# Autodesk Inventor assembly: GPS-Compass_assembly
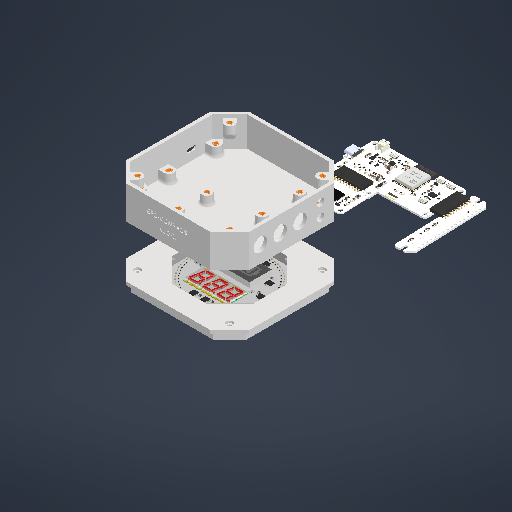
[picture p0: Inventor's stored thumbnail of the model, 512x512]
Saved by Autodesk Inventor 2026.1 (Build 301233020, 233B)
## iProperties
Created: 2025-11-19
Part Number: GPS-Compass_assembly
Document SubType Name: Assembly
Designer: MenMe
Author: MenMe
## Documents named in this file (10)
- C:\Users\MenMe\Documents\GitHub\GPS-Compass\Mechanical\GPS-Compass_assembly\GPS-Compass_assembly.iam
- C:\Users\MenMe\Documents\GitHub\GPS-Compass\Mechanical\GPS-Compass_assembly\GPS-Compass_box.ipt
- C:\Users\MenMe\Documents\GitHub\GPS-Compass\Mechanical\GPS-Compass_assembly\GPS-Compass_top.ipt
- C:\Users\MenMe\Documents\GitHub\GPS-Compass\Mechanical\PCB_3D_models\GPS-Compass_Arrow\GPS-Compass_Arrow\GPS-Compass_Arrow.iam
- C:\Users\MenMe\Documents\GitHub\GPS-Compass\Mechanical\GPS-Compass_assembly\GPS-Compass_plexi.ipt
- C:\Users\MenMe\Documents\GitHub\GPS-Compass\Mechanical\GPS-Compass_assembly\DODGE INSERT M3X4(D5-Dill4.8)\DODGE INSERT M3X4(D5-Dill4.8)\DODGE INSERT M3X4(D5-Dill4.8).ipt
- C:\Users\MenMe\Documents\Inventor\Content Center Files\R2026\en-US\ISO 4762(2)\ISO 4762 - M3 x 16ISO.ipt
- C:\Users\MenMe\Documents\GitHub\GPS-Compass\Mechanical\PCB_3D_models\GPS-Compass\GPS-Compass\GPS-Compass.ipt
- C:\Users\MenMe\Documents\GitHub\GPS-Compass\Mechanical\PCB_3D_models\GPS-Compass_UI\GPS-Compass_UI\GPS-Compass_UI.ipt
- C:\Users\MenMe\Documents\GitHub\GPS-Compass\Mechanical\GPS-Compass_GNSS\GPS-Compass_GNSS\GPS-Compass_GNSS.iam
## Components (24 placed, 9 different names)
1. GPS-Compass_box:1 — Mate:2, Mate:3, Mate:4, Insert:1, Insert:6, Insert:7, Insert:8, Insert:9, Mate:11, Insert:10, Insert:11, Insert:12, Insert:13, Insert:14, Insert:15, Insert:16
2. GPS-Compass_top:1 — Mate:2, Mate:3, Mate:4, Mate:5, Mate:6, Mate:7, Mate:8, Mate:9, Mate:10, Insert:2, Insert:3, Insert:4, Insert:5
3. GPS-Compass_Arrow:1 [sub-assembly] — Mate:5, Mate:6, Mate:7
4. GPS-Compass_plexi:1 — Mate:8, Mate:9, Mate:10
5. DODGE INSERT M3X4(D5-Dill4.8):1 — Insert:1
6. DODGE INSERT M3X4(D5-Dill4.8):2 — Insert:6
7. ISO 4762 M3 x 16:1 — Insert:2
8. ISO 4762 M3 x 16:2 — Insert:3
9. ISO 4762 M3 x 16:3 — Insert:4
10. ISO 4762 M3 x 16:4 — Insert:5
11. DODGE INSERT M3X4(D5-Dill4.8):3 — Insert:7
12. DODGE INSERT M3X4(D5-Dill4.8):4 — Insert:8
13. DODGE INSERT M3X4(D5-Dill4.8):5 — Insert:9
14. DODGE INSERT M3X4(D5-Dill4.8):6 — Mate:11
15. DODGE INSERT M3X4(D5-Dill4.8):7 — Insert:10
16. DODGE INSERT M3X4(D5-Dill4.8):8 — Insert:11
17. DODGE INSERT M3X4(D5-Dill4.8):9 — Insert:12
18. DODGE INSERT M3X4(D5-Dill4.8):10 — Insert:13
19. DODGE INSERT M3X4(D5-Dill4.8):11 — Insert:14
20. DODGE INSERT M3X4(D5-Dill4.8):12 — Insert:15
21. GPS-Compass:1 — Mate:13, Flush:3, Flush:4, Flush:5, Mate:14, Flush:6
22. DODGE INSERT M3X4(D5-Dill4.8):13 — Insert:16
23. GPS-Compass_UI:1 — Mate:13, Flush:3, Flush:6
24. GPS-Compass_GNSS:1 [sub-assembly] — Flush:4, Flush:5, Mate:14
## Relationships (32: Insert 16, Mate 12, Flush 4)
- Mate:2 (-80 mm): GPS-Compass_box:1 ↔ GPS-Compass_top:1
- Mate:3: GPS-Compass_box:1 ↔ GPS-Compass_top:1
- Mate:4: GPS-Compass_box:1 ↔ GPS-Compass_top:1
- Mate:5: GPS-Compass_top:1 ↔ GPS-Compass_Arrow:1
- Mate:6: GPS-Compass_top:1 ↔ GPS-Compass_Arrow:1
- Mate:7: GPS-Compass_top:1 ↔ GPS-Compass_Arrow:1
- Mate:8: GPS-Compass_top:1 ↔ GPS-Compass_plexi:1
- Mate:9: GPS-Compass_top:1 ↔ GPS-Compass_plexi:1
- Mate:10: GPS-Compass_top:1 ↔ GPS-Compass_plexi:1
- Insert:1: GPS-Compass_box:1 ↔ DODGE INSERT M3X4(D5-Dill4.8):1
- Insert:2: GPS-Compass_top:1 ↔ ISO 4762 M3 x 16:1
- Insert:3: GPS-Compass_top:1 ↔ ISO 4762 M3 x 16:2
- Insert:4: GPS-Compass_top:1 ↔ ISO 4762 M3 x 16:3
- Insert:5: GPS-Compass_top:1 ↔ ISO 4762 M3 x 16:4
- Insert:6: GPS-Compass_box:1 ↔ DODGE INSERT M3X4(D5-Dill4.8):2
- Insert:7: GPS-Compass_box:1 ↔ DODGE INSERT M3X4(D5-Dill4.8):3
- Insert:8: GPS-Compass_box:1 ↔ DODGE INSERT M3X4(D5-Dill4.8):4
- Insert:9: GPS-Compass_box:1 ↔ DODGE INSERT M3X4(D5-Dill4.8):5
- Mate:11: GPS-Compass_box:1 ↔ DODGE INSERT M3X4(D5-Dill4.8):6
- Insert:10: GPS-Compass_box:1 ↔ DODGE INSERT M3X4(D5-Dill4.8):7
- Insert:11: GPS-Compass_box:1 ↔ DODGE INSERT M3X4(D5-Dill4.8):8
- Insert:12: GPS-Compass_box:1 ↔ DODGE INSERT M3X4(D5-Dill4.8):9
- Insert:13: GPS-Compass_box:1 ↔ DODGE INSERT M3X4(D5-Dill4.8):10
- Insert:14: GPS-Compass_box:1 ↔ DODGE INSERT M3X4(D5-Dill4.8):11
- Insert:15: GPS-Compass_box:1 ↔ DODGE INSERT M3X4(D5-Dill4.8):12
- Insert:16: GPS-Compass_box:1 ↔ DODGE INSERT M3X4(D5-Dill4.8):13
- Mate:13: GPS-Compass:1 ↔ GPS-Compass_UI:1
- Flush:3: GPS-Compass:1 ↔ GPS-Compass_UI:1
- Flush:4: GPS-Compass:1 ↔ GPS-Compass_GNSS:1
- Flush:5: GPS-Compass:1 ↔ GPS-Compass_GNSS:1
- Mate:14: GPS-Compass:1 ↔ GPS-Compass_GNSS:1
- Flush:6: GPS-Compass:1 ↔ GPS-Compass_UI:1
